# Autodesk Inventor assembly: battery holder
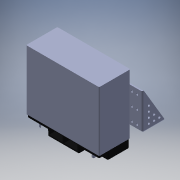
[picture p0: Inventor's stored thumbnail of the model, 180x180]
Saved by Autodesk Inventor 2016 (Build 200138000, 138)
## iProperties
Created: 2016-02-08
Part Number: battery holder
Document SubType Name: Assembly
Designer: gus
Mass: 2218.31 g
Surface Area: 1575.43 cm^2
Volume: 2218.31 cm^3
Density: 1 g/cm^3
Author: gus
## Documents named in this file (5)
- \\Mac\Home\Desktop\1510-stronghold-CAD-master\shooter\battery holder.iam
- \\Mac\Home\Desktop\1510-stronghold-CAD-master\shooter\plate.ipt
- \\Mac\Home\Desktop\1510-stronghold-CAD-master\batterystuff\User Library-Battery-6.ipt
- \\Mac\Home\Desktop\1510-stronghold-CAD-master\idler pully for pickerupthingy\battery plate.ipt
- \\Mac\Home\Desktop\1510-stronghold-CAD-master\batterystuff\battery corner.ipt
## Components (6 placed, 4 different names)
1. plate:1
2. User Library-Battery-6:1 — Mate:2, Flush:3, Mate:7, Mate:8, Mate:9
3. plate:2 — Mate:2, Flush:3
4. battery plate:1 — Flush:4, Mate:3, Flush:5, Mate:4, Mate:5, Mate:6, Mate:7
5. battery corner:1 — Flush:4, Mate:3, Flush:5, Mate:9
6. battery corner:2 — Mate:4, Mate:5, Mate:6, Mate:8
## Relationships (11: Mate 8, Flush 3)
- Mate:2: User Library-Battery-6:1 ↔ plate:2
- Flush:3 (25.4 mm): User Library-Battery-6:1 ↔ plate:2
- Flush:4: battery plate:1 ↔ battery corner:1
- Mate:3: battery plate:1 ↔ battery corner:1
- Flush:5: battery plate:1 ↔ battery corner:1
- Mate:4: battery plate:1 ↔ battery corner:2
- Mate:5: battery plate:1 ↔ battery corner:2
- Mate:6: battery plate:1 ↔ battery corner:2
- Mate:7: User Library-Battery-6:1 ↔ battery plate:1
- Mate:8: User Library-Battery-6:1 ↔ battery corner:2
- Mate:9: User Library-Battery-6:1 ↔ battery corner:1
